# Autodesk Inventor assembly: wheel4_MIR1
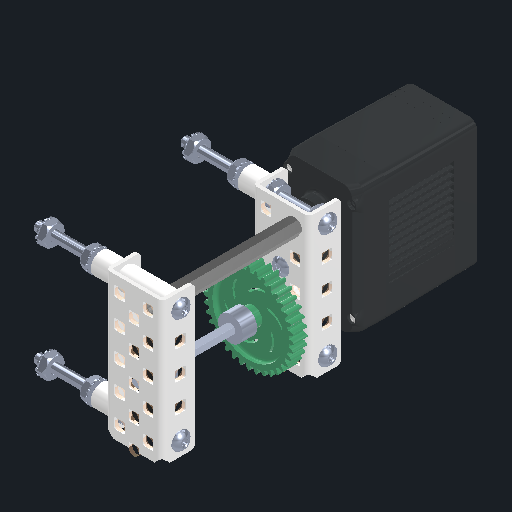
[picture p0: Inventor's stored thumbnail of the model, 512x512]
Saved by Autodesk Inventor 2024 (Build 280153000, 153)
## iProperties
Created: 2023-08-09
Part Number: wheel4_MIR1
Document SubType Name: Assembly
Designer: macbook
Author: macbook
## Documents named in this file (21)
- \\Mac\Home\Desktop\code\7899V-VRC-OVER-UNDER\Cad\VEX-CAD-Inventor-1.4.0\Assembly\v0.2\wheel4_MIR1.iam
- \\Mac\Home\Desktop\code\7899V-VRC-OVER-UNDER\Cad\VEX-CAD-Inventor-1.4.0\Motion\Gears\LS 36T Gear_MIR2.ipt
- \\Mac\Home\Desktop\code\7899V-VRC-OVER-UNDER\Cad\VEX-CAD-Inventor-1.4.0\Motion\Shaft LS\Bearing Flat_MIR2.ipt
- \\Mac\Home\Desktop\code\7899V-VRC-OVER-UNDER\Cad\VEX-CAD-Inventor-1.4.0\Motion\Shaft LS\Shaft LS\Shaft LS 3.5.ipt
- \\Mac\Home\Desktop\code\7899V-VRC-OVER-UNDER\Cad\VEX-CAD-Inventor-1.4.0\Motion\Shaft LS\Shaft LS.ipt
- \\Mac\Home\Desktop\code\7899V-VRC-OVER-UNDER\Cad\VEX-CAD-Inventor-1.4.0\Motion\Shaft LS\Shaft Collar Metal\Shaft Collar Set Screw_MIR1.iam
- \\Mac\Home\Desktop\code\7899V-VRC-OVER-UNDER\Cad\VEX-CAD-Inventor-1.4.0\Electronics\Motors with Screws\AluM-StarS_MIR2.iam
- \\Mac\Home\Desktop\code\7899V-VRC-OVER-UNDER\Cad\VEX-CAD-Inventor-1.4.0\Motion\Spacers\Spacer Nylon .500 OD\NSpacer White .500 OD x .375.ipt
- \\Mac\Home\Desktop\code\7899V-VRC-OVER-UNDER\Cad\VEX-CAD-Inventor-1.4.0\Motion\Spacers\Spacer Nylon .500 OD.ipt
- \\Mac\Home\Desktop\code\7899V-VRC-OVER-UNDER\Cad\VEX-CAD-Inventor-1.4.0\Motion\Spacers\Spacer Nylon .500 OD\NSpacer White .500 OD x .250.ipt
- \\Mac\Home\Desktop\code\7899V-VRC-OVER-UNDER\Cad\VEX-CAD-Inventor-1.4.0\Structure\C Channel\Aluminum 1x2x1\Alu C 1x2x1x5_MIR2.ipt
- \\Mac\Home\Desktop\code\7899V-VRC-OVER-UNDER\Cad\VEX-CAD-Inventor-1.4.0\Structure\Hardware\Nut Keps_MIR1.ipt
- \\Mac\Home\Desktop\code\7899V-VRC-OVER-UNDER\Cad\VEX-CAD-Inventor-1.4.0\Motion\Spacers\Spacer Nylon .313 OD\NSpacer .313 OD x .375.ipt
- \\Mac\Home\Desktop\code\7899V-VRC-OVER-UNDER\Cad\VEX-CAD-Inventor-1.4.0\Motion\Spacers\Spacer Nylon .313 OD.ipt
- \\Mac\Home\Desktop\code\7899V-VRC-OVER-UNDER\Cad\VEX-CAD-Inventor-1.4.0\Motion\Spacers\Spacer Nylon .313 OD\NSpacer .313 OD x .500.ipt
- \\Mac\Home\Desktop\code\7899V-VRC-OVER-UNDER\Cad\VEX-CAD-Inventor-1.4.0\Structure\Hardware\Screw Steel - Star\SScrew Star Smooth 2.500.ipt
- \\Mac\Home\Desktop\code\7899V-VRC-OVER-UNDER\Cad\VEX-CAD-Inventor-1.4.0\Structure\Hardware\Screw Steel - Star.ipt
- \\Mac\Home\Desktop\code\7899V-VRC-OVER-UNDER\Cad\VEX-CAD-Inventor-1.4.0\Structure\Hardware\Screw Steel - Star\SScrew Star Smooth 1.750.ipt
- \\Mac\Home\Desktop\code\7899V-VRC-OVER-UNDER\Cad\VEX-CAD-Inventor-1.4.0\Structure\Hardware\Nut Thin Nylock_MIR2.ipt
- \\Mac\Home\Desktop\code\7899V-VRC-OVER-UNDER\Cad\VEX-CAD-Inventor-1.4.0\Structure\Standoff\Standoff 2.50.ipt
- \\Mac\Home\Desktop\code\7899V-VRC-OVER-UNDER\Cad\VEX-CAD-Inventor-1.4.0\Structure\Standoff.ipt
## Components (34 placed, 15 different names)
1. LS 36T Gear_MIR2:1 — Insert:2, Insert:1
2. Bearing Flat_MIR2:1 — Insert:5, Insert:4, Insert:10, Cylindrical:1
3. Shaft LS 3.5:1 — Mate:1, Cylindrical:1, Cylindrical:2
4. Shaft Collar Set Screw_MIR1:1 [sub-assembly] — Insert:5
5. Shaft Collar Set Screw_MIR1:2 [sub-assembly] — Insert:2, Cylindrical:2
6. AluM-StarS_MIR2:1 [sub-assembly] — Mate:1, Insert:4
7. NSpacer White .500 OD x .375:1 — Insert:12, Insert:3
8. NSpacer White .500 OD x .250:2 — Insert:3, Insert:1
9. Alu C 1x2x1x5_MIR2:1 — Insert:12, Insert:13, Insert:16, Insert:17, Insert:21, Insert:23, Insert:24, Insert:29, Insert:34, Insert:38
10. Alu C 1x2x1x5_MIR2:2 — Insert:13, Insert:10, Insert:14, Insert:15, Insert:20, Insert:22, Insert:25, Insert:26, Insert:35, Insert:39
11. Nut Keps_MIR1:1 — Insert:14
12. Nut Keps_MIR1:2 — Insert:15
13. Nut Keps_MIR1:3 — Insert:16
14. Nut Keps_MIR1:4 — Insert:17
15. NSpacer .313 OD x .375:1 — Insert:18
16. NSpacer .313 OD x .500:2 — Insert:20, Insert:18
17. NSpacer .313 OD x .375:3 — Insert:19
18. NSpacer .313 OD x .500:4 — Insert:21, Insert:19
19. NSpacer .313 OD x .375:5 — Insert:22, Insert:27
20. NSpacer .313 OD x .375:6 — Insert:23, Insert:36
21. NSpacer .313 OD x .375:7 — Insert:25, Insert:37
22. NSpacer .313 OD x .375:8 — Insert:24, Insert:30
23. SScrew Star Smooth 2.500:1 — Insert:26
24. Nut Keps_MIR1:5 — Insert:27, Insert:28
25. Nut Keps_MIR1:6 — Insert:28
26. SScrew Star Smooth 1.750:2 — Insert:29
27. Nut Thin Nylock_MIR2:1 — Insert:30
28. Nut Keps_MIR1:7 — Insert:36, Insert:31
29. Nut Keps_MIR1:8 — Insert:31
30. SScrew Star Smooth 2.500:3 — Insert:35
31. SScrew Star Smooth 2.500:4 — Insert:34
32. Nut Keps_MIR1:9 — Insert:37, Insert:33
33. Nut Keps_MIR1:10 — Insert:33
34. Standoff 2.50:1 — Insert:39, Insert:38
## Relationships (36: Insert 33, CylindricalJoint 2, Mate 1)
- Insert:5: Bearing Flat_MIR2:1 ↔ Shaft Collar Set Screw_MIR1:1
- Insert:2: LS 36T Gear_MIR2:1 ↔ Shaft Collar Set Screw_MIR1:2
- Mate:1: Shaft LS 3.5:1 ↔ AluM-StarS_MIR2:1
- Insert:4 (59.5312 mm): Bearing Flat_MIR2:1 ↔ AluM-StarS_MIR2:1
- Insert:12: NSpacer White .500 OD x .375:1 ↔ Alu C 1x2x1x5_MIR2:1
- Insert:13 (63.5 mm): Alu C 1x2x1x5_MIR2:1 ↔ Alu C 1x2x1x5_MIR2:2
- Insert:10: Bearing Flat_MIR2:1 ↔ Alu C 1x2x1x5_MIR2:2
- Insert:14: Alu C 1x2x1x5_MIR2:2 ↔ Nut Keps_MIR1:1
- Insert:15: Alu C 1x2x1x5_MIR2:2 ↔ Nut Keps_MIR1:2
- Insert:16: Alu C 1x2x1x5_MIR2:1 ↔ Nut Keps_MIR1:3
- Insert:17: Alu C 1x2x1x5_MIR2:1 ↔ Nut Keps_MIR1:4
- Insert:20: Alu C 1x2x1x5_MIR2:2 ↔ NSpacer .313 OD x .500:2
- Insert:18: NSpacer .313 OD x .375:1 ↔ NSpacer .313 OD x .500:2
- Insert:21: Alu C 1x2x1x5_MIR2:1 ↔ NSpacer .313 OD x .500:4
- Insert:19: NSpacer .313 OD x .375:3 ↔ NSpacer .313 OD x .500:4
- Insert:22: Alu C 1x2x1x5_MIR2:2 ↔ NSpacer .313 OD x .375:5
- Insert:23: Alu C 1x2x1x5_MIR2:1 ↔ NSpacer .313 OD x .375:6
- Insert:25: Alu C 1x2x1x5_MIR2:2 ↔ NSpacer .313 OD x .375:7
- Insert:24: Alu C 1x2x1x5_MIR2:1 ↔ NSpacer .313 OD x .375:8
- Insert:26: Alu C 1x2x1x5_MIR2:2 ↔ SScrew Star Smooth 2.500:1
- Insert:27 (1.5875 mm): NSpacer .313 OD x .375:5 ↔ Nut Keps_MIR1:5
- Insert:28 (15.24 mm): Nut Keps_MIR1:5 ↔ Nut Keps_MIR1:6
- Insert:29: Alu C 1x2x1x5_MIR2:1 ↔ SScrew Star Smooth 1.750:2
- Insert:36 (1.5875 mm): NSpacer .313 OD x .375:6 ↔ Nut Keps_MIR1:7
- Insert:31 (15.24 mm): Nut Keps_MIR1:7 ↔ Nut Keps_MIR1:8
- Insert:35: Alu C 1x2x1x5_MIR2:2 ↔ SScrew Star Smooth 2.500:3
- Insert:34: Alu C 1x2x1x5_MIR2:1 ↔ SScrew Star Smooth 2.500:4
- Insert:37 (1.5875 mm): NSpacer .313 OD x .375:7 ↔ Nut Keps_MIR1:9
- Insert:33 (15.24 mm): Nut Keps_MIR1:9 ↔ Nut Keps_MIR1:10
- Insert:30 (1.5875 mm): NSpacer .313 OD x .375:8 ↔ Nut Thin Nylock_MIR2:1
- Insert:3 (1.5875 mm): NSpacer White .500 OD x .375:1 ↔ NSpacer White .500 OD x .250:2
- Insert:1: LS 36T Gear_MIR2:1 ↔ NSpacer White .500 OD x .250:2
- Insert:39: Alu C 1x2x1x5_MIR2:2 ↔ Standoff 2.50:1
- Insert:38: Alu C 1x2x1x5_MIR2:1 ↔ Standoff 2.50:1
- Cylindrical:1: Bearing Flat_MIR2:1 ↔ Shaft LS 3.5:1
- Cylindrical:2: Shaft LS 3.5:1 ↔ Shaft Collar Set Screw_MIR1:2
